# Autodesk Inventor assembly: Assembly
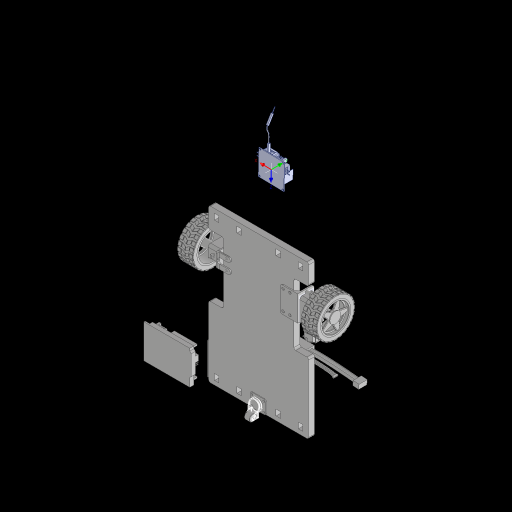
[picture p0: Inventor's stored thumbnail of the model, 512x512]
Saved by Autodesk Inventor 2024.3 (Build 283343010, 343A)
## iProperties
Created: 2025-04-09
Part Number: Assembly
Document SubType Name: Assembly
Designer: Oleg Kelner
Author: Oleg Kelner
## Documents named in this file (11)
- D:\Study\Prototyping\Prototyping-SS25-Team-C4\3DModels\Assembly.iam
- D:\Study\Prototyping\Prototyping-SS25-Team-C4\3DModels\Basic components\chassis.ipt
- D:\Study\Prototyping\Prototyping-SS25-Team-C4\3DModels\Basic components\motor-with-tire.ipt
- D:\Study\Prototyping\Prototyping-SS25-Team-C4\3DModels\Oleg's details\motorHolder_MIR.ipt
- D:\Study\Prototyping\Prototyping-SS25-Team-C4\3DModels\Basic components\front-wheel.ipt
- D:\Study\Prototyping\Prototyping-SS25-Team-C4\3DModels\Basic components\motor-with-tire_MIR.ipt
- D:\Study\Prototyping\Prototyping-SS25-Team-C4\3DModels\Basic components\lipo-battery.ipt
- D:\Study\Prototyping\Prototyping-SS25-Team-C4\3DModels\Basic components\arduino.ipt
- D:\Study\Prototyping\Prototyping-SS25-Team-C4\3DModels\Basic components\breadboard.ipt
- D:\Study\Prototyping\Prototyping-SS25-Team-C4\3DModels\Basic components\motorcontroler.ipt
- D:\Study\Prototyping\Prototyping-SS25-Team-C4\3DModels\Oleg's details\vertMotorHolder.ipt
## Components (10 placed, 10 different names)
1. chassis:1 — Angle:1, Planar:2, Mate:1, Mate:2, Flush:1, Rigid:1, Planar:3, Angle:2, Planar:4, Angle:3, Planar:5, Angle:4, Planar:6, Angle:5
2. motor-with-tire:1 — Rotational:4, Tangent:1, Rotational:5, Insert:1
3. motorHolder_MIR:1 — Rotational:4, Rotational:5, Planar:2, Mate:1, Mate:2
4. front-wheel:1 — Rigid:1
5. motor-with-tire_MIR:1 — Tangent:3, Insert:1, Angle:5, Flush:2, Flush:3, Rigid:2
6. lipo-battery:1 — Planar:3, Angle:2
7. arduino:1 — Planar:5, Angle:4
8. breadboard:1 — Planar:4, Angle:3
9. motorcontroler:1 — Planar:6
10. vertMotorHolder:1 — Flush:2, Flush:3, Rigid:2
## Relationships (22: Angle 5, PlanarJoint 5, Flush 3, RevoluteJoint 2, Tangent 2, Mate 2, WeldJoint 2, Insert 1)
- Rotational:4 [RevoluteJoint]: motor-with-tire:1 ↔ motorHolder_MIR:1
- Angle:1 (0 deg): chassis:1
- Tangent:1: motor-with-tire:1
- Rotational:5 [RevoluteJoint]: motor-with-tire:1 ↔ motorHolder_MIR:1
- Planar:2: chassis:1 ↔ motorHolder_MIR:1
- Mate:1 (-21.5 mm): chassis:1 ↔ motorHolder_MIR:1
- Mate:2 (18 mm): chassis:1 ↔ motorHolder_MIR:1
- Flush:1 (-85 mm): chassis:1
- Tangent:3: motor-with-tire_MIR:1
- Rigid:1 [WeldJoint]: chassis:1 ↔ front-wheel:1
- Planar:3: chassis:1 ↔ lipo-battery:1
- Angle:2 (0 deg): chassis:1 ↔ lipo-battery:1
- Planar:4: chassis:1 ↔ breadboard:1
- Angle:3 (0 deg): chassis:1 ↔ breadboard:1
- Planar:5: chassis:1 ↔ arduino:1
- Angle:4 (0 deg): chassis:1 ↔ arduino:1
- Planar:6: chassis:1 ↔ motorcontroler:1
- Insert:1 (120.14 mm): motor-with-tire:1 ↔ motor-with-tire_MIR:1
- Angle:5 (-90 deg): chassis:1 ↔ motor-with-tire_MIR:1
- Flush:2: motor-with-tire_MIR:1 ↔ vertMotorHolder:1
- Flush:3: motor-with-tire_MIR:1 ↔ vertMotorHolder:1
- Rigid:2 [WeldJoint]: motor-with-tire_MIR:1 ↔ vertMotorHolder:1
